# Autodesk Inventor assembly: WheelAndFlywheel2
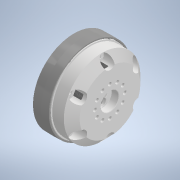
[picture p0: Inventor's stored thumbnail of the model, 180x180]
Saved by Autodesk Inventor 2020 (Build 240168000, 168)
## iProperties
Created: 2020-02-08
Part Number: WheelAndFlywheel2
Document SubType Name: Assembly
Designer: srini
Author: srini
## Documents named in this file (6)
- C:\Users\srini\Documents\FRC\2020\Shooter\WheelAndFlywheel2.iam
- C:\Users\srini\Documents\FRC\2020\6 wheel Rev 4.ipt
- C:\Users\srini\Documents\FRC\2020\Shooter\WheelInsertFlywheelTry2.ipt
- C:\Users\srini\Documents\FRC\2020\Shooter\TopFlywheelClamp2.ipt
- C:\Users\srini\Documents\FRC\2020\Shooter\Flywheel.ipt
- C:\Users\srini\Documents\FRC\2020\Shooter\WheelClampBottomB.ipt
## Components (5 placed, 5 different names)
1. 6 wheel Rev 4:1 — Mate:1, Flush:1, Mate:2, Mate:3, Flush:2, Mate:6, Mate:8
2. WheelInsertFlywheelTry2:1 — Flush:2, Mate:7, Flush:3
3. TopFlywheelClamp2:1 — Insert:1, Mate:8
4. Flywheel:1 — Mate:6, Insert:1, Mate:7
5. WheelClampBottomB:1 — Flush:3
## Relationships (13: Mate 8, Flush 3, Angle 1, Insert 1)
- Mate:1: 6 wheel Rev 4:1
- Flush:1 (-1.27 mm): 6 wheel Rev 4:1
- Mate:2: 6 wheel Rev 4:1
- Mate:3: 6 wheel Rev 4:1
- Mate:4
- Mate:5
- Angle:1 (0 deg)
- Flush:2: 6 wheel Rev 4:1 ↔ WheelInsertFlywheelTry2:1
- Mate:6: 6 wheel Rev 4:1 ↔ Flywheel:1
- Insert:1: TopFlywheelClamp2:1 ↔ Flywheel:1
- Mate:7: WheelInsertFlywheelTry2:1 ↔ Flywheel:1
- Mate:8: 6 wheel Rev 4:1 ↔ TopFlywheelClamp2:1
- Flush:3: WheelInsertFlywheelTry2:1 ↔ WheelClampBottomB:1
